# Autodesk Inventor assembly: UpperBackLink
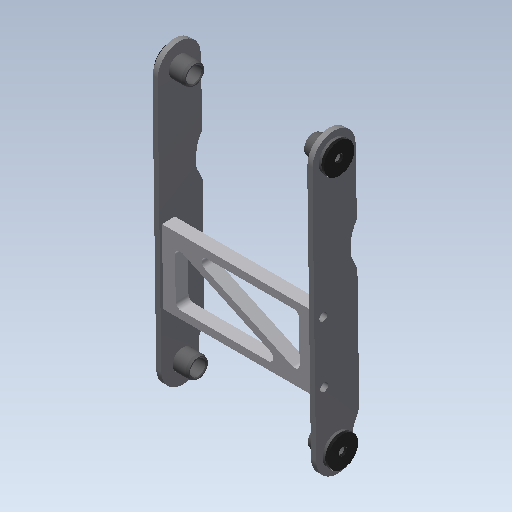
[picture p0: Inventor's stored thumbnail of the model, 512x512]
Saved by Autodesk Inventor 2020 (Build 240168000, 168)
## iProperties
Created: 2016-08-23
Part Number: UpperBackLink
Material: 一般
Document SubType Name: Assembly
Designer: hiro
Mass: 25.265 g
Surface Area: 146.992 cm^2
Volume: 11.3922 cm^3
Density: 2.21774 g/cm^3
Author: hiro
## Documents named in this file (5)
- C:\Users\Masato\Desktop\最新版\OpenPlatform_ver3_0\下半身\リンク\UpperBackLink.iam
- C:\Users\Masato\Desktop\最新版\OpenPlatform_ver3_0\下半身\リンク\リンク_メインフレーム_6_1.ipt
- C:\Users\Masato\Desktop\最新版\OpenPlatform_ver3_0\下半身\リンク\リンク_ふくらはぎ_サブフレーム_1_2.ipt
- C:\Users\Masato\Desktop\最新版\OpenPlatform_ver3_0\Ready_Made\80F-0608.ipt
- C:\Users\Masato\Desktop\最新版\OpenPlatform_ver3_0\Ready_Made\UUW-0312-10BH.ipt
## Components (11 placed, 4 different names)
1. リンク_ふくらはぎ_サブフレーム_1_2(予備案):1 — 挿入:2, 挿入:4, 挿入:11, 挿入:12
2. リンク_メインフレーム_6_1:1 — 挿入:2, 挿入:11, 挿入:14, 挿入:16
3. リンク_メインフレーム_6_1:2 — 挿入:4, 挿入:12, 挿入:13, 挿入:15
4. 80F-0608:1 — 挿入:13, 挿入:20
5. 80F-0608:2 — 挿入:14, 挿入:18
6. 80F-0608:3 — 挿入:15, 挿入:19
7. 80F-0608:4 — 挿入:16, 挿入:17
8. UUW-0312-10BH:1 — 挿入:17
9. UUW-0312-10BH:2 — 挿入:18
10. UUW-0312-10BH:3 — 挿入:20
11. UUW-0312-10BH:4 — 挿入:19
## Relationships (12: Insert 12)
- 挿入:2 [Insert]: リンク_ふくらはぎ_サブフレーム_1_2(予備案):1 ↔ リンク_メインフレーム_6_1:1
- 挿入:4 [Insert]: リンク_ふくらはぎ_サブフレーム_1_2(予備案):1 ↔ リンク_メインフレーム_6_1:2
- 挿入:11 [Insert]: リンク_ふくらはぎ_サブフレーム_1_2(予備案):1 ↔ リンク_メインフレーム_6_1:1
- 挿入:12 [Insert]: リンク_ふくらはぎ_サブフレーム_1_2(予備案):1 ↔ リンク_メインフレーム_6_1:2
- 挿入:13 [Insert]: リンク_メインフレーム_6_1:2 ↔ 80F-0608:1
- 挿入:14 [Insert]: リンク_メインフレーム_6_1:1 ↔ 80F-0608:2
- 挿入:15 [Insert]: リンク_メインフレーム_6_1:2 ↔ 80F-0608:3
- 挿入:16 [Insert]: リンク_メインフレーム_6_1:1 ↔ 80F-0608:4
- 挿入:17 [Insert]: 80F-0608:4 ↔ UUW-0312-10BH:1
- 挿入:18 [Insert]: 80F-0608:2 ↔ UUW-0312-10BH:2
- 挿入:19 [Insert]: 80F-0608:3 ↔ UUW-0312-10BH:4
- 挿入:20 [Insert]: 80F-0608:1 ↔ UUW-0312-10BH:3
